# Autodesk Inventor assembly: NewExhaustValve
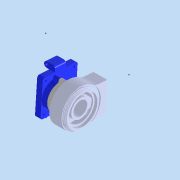
[picture p0: Inventor's stored thumbnail of the model, 180x180]
Saved by Autodesk Inventor 2020 (Build 240168000, 168)
## iProperties
Created: 2020-04-10
Part Number: NewExhaustValve
Document SubType Name: Assembly
Designer: Simon
Author: Simon
## Documents named in this file (3)
- D:\GrabCAD\MTL Ventilator Design\Filter housing with o ring\NewExhaustValve.iam
- D:\GrabCAD\MTL Ventilator Design\Filter housing with o ring\new_PEEP_valve.ipt
- D:\GrabCAD\MTL Ventilator Design\Filter housing with o ring\Exhaust_filter_bottom.ipt
## Components (2 placed, 2 different names)
1. new_PEEP_valve:1 — Mate:1, Angle:1, Mate:2
2. Exhaust_filter_bottom:1 — Mate:1, Angle:1, Mate:2
## Relationships (3: Mate 2, Angle 1)
- Mate:1: new_PEEP_valve:1 ↔ Exhaust_filter_bottom:1
- Angle:1 (0 deg): new_PEEP_valve:1 ↔ Exhaust_filter_bottom:1
- Mate:2: new_PEEP_valve:1 ↔ Exhaust_filter_bottom:1
